# Autodesk Inventor assembly: v2_obstaculo
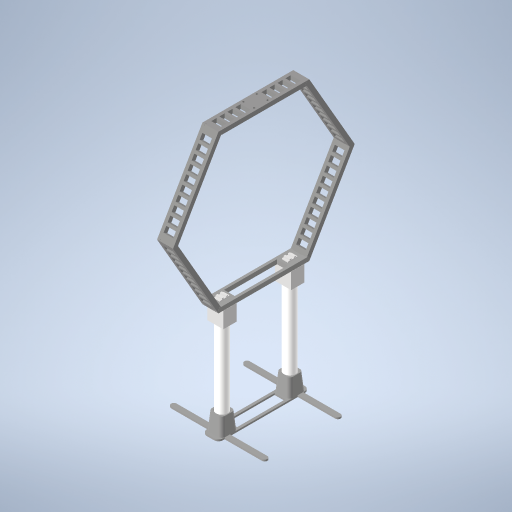
[picture p0: Inventor's stored thumbnail of the model, 512x512]
Saved by Autodesk Inventor 2024.3 (Build 283343000, 343)
## iProperties
Created: 2024-10-22
Part Number: v2_obstaculo
Document SubType Name: Assembly
Designer: pjcaa
Author: pjcaa
## Documents named in this file (8)
- C:\Users\pjcaa\Desktop\Educación\Semestres\5to año - Semestre 10\Diseño e innovación en ingeniería 2\Trabajo de graduacion\Archivos CAD\OBSTACULO_HEXAGONAL\ENSAMBLE_CON_EXTENSION.iam
- C:\Users\pjcaa\Desktop\Educación\Semestres\5to año - Semestre 10\Diseño e innovación en ingeniería 2\Trabajo de graduacion\Archivos CAD\OBSTACULO_HEXAGONAL\HEXAGONO_BASE.ipt
- C:\Users\pjcaa\Desktop\Educación\Semestres\5to año - Semestre 10\Diseño e innovación en ingeniería 2\Trabajo de graduacion\Archivos CAD\OBSTACULO_HEXAGONAL\EXTENSION_SOPORTE.ipt
- C:\Users\pjcaa\Desktop\Educación\Semestres\5to año - Semestre 10\Diseño e innovación en ingeniería 2\Trabajo de graduacion\Archivos CAD\OBSTACULO_HEXAGONAL\PIN.ipt
- C:\Users\pjcaa\Desktop\Educación\Semestres\5to año - Semestre 10\Diseño e innovación en ingeniería 2\Trabajo de graduacion\Archivos CAD\OBSTACULO_HEXAGONAL\EXTENSION_BASE.ipt
- C:\Users\pjcaa\Desktop\Educación\Semestres\5to año - Semestre 10\Diseño e innovación en ingeniería 2\Trabajo de graduacion\Archivos CAD\OBSTACULO_HEXAGONAL\HEXAGONO_LATERAL.ipt
- C:\Users\pjcaa\Desktop\Educación\Semestres\5to año - Semestre 10\Diseño e innovación en ingeniería 2\Trabajo de graduacion\Archivos CAD\OBSTACULO_HEXAGONAL\HEXGAONO_SUPERIOR.ipt
- C:\Users\pjcaa\Desktop\Educación\Semestres\5to año - Semestre 10\Diseño e innovación en ingeniería 2\Trabajo de graduacion\Archivos CAD\OBSTACULO_HEXAGONAL\TUBO.ipt
## Components (13 placed, 5 different names)
1. HEXAGONO_BASE:1 — Mate:1, Mate:2, Mate:3, Mate:4, Mate:5, Mate:10, Flush:7, Flush:8, Flush:9, Flush:10, Mate:11
2. sujetador_base:1 — Mate:1, Flush:1, Flush:2, Mate:2, Mate:6, Mate:7, Mate:14, Mate:18
3. sujetador_base:2 — Flush:1, Flush:2, Mate:3, Mate:4, Mate:13, Mate:19
4. sujetador_base:3 — Mate:5, Mate:6, Mate:7, Flush:14, Flush:15
5. EXTENSION_BASE:1 — Mate:13, Mate:14, Mate:15, Mate:16, Mate:17
6. HEXAGONO_LATERAL:1 — Mate:8, Flush:3, Flush:4, Flush:10, Mate:11
7. HEXGAONO_SUPERIOR:1 — Mate:12, Flush:11, Flush:12
8. HEXAGONO_LATERAL:2 — Mate:8, Flush:3, Flush:4, Flush:9, Mate:12, Flush:11
9. HEXAGONO_LATERAL:3 — Mate:10, Flush:7, Flush:8
10. HEXAGONO_LATERAL:4 — Flush:12
11. sujetador_base:4 — Mate:16, Flush:13, Mate:17, Mate:18
12. sujetador_base:5 — Mate:15, Flush:13
13. sujetador_base:6 — Flush:14, Flush:15, Mate:19
## Relationships (34: Mate 19, Flush 15)
- Mate:1: HEXAGONO_BASE:1 ↔ sujetador_base:1
- Flush:1: sujetador_base:1 ↔ sujetador_base:2
- Flush:2: sujetador_base:1 ↔ sujetador_base:2
- Mate:2: HEXAGONO_BASE:1 ↔ sujetador_base:1
- Mate:3: HEXAGONO_BASE:1 ↔ sujetador_base:2
- Mate:4: HEXAGONO_BASE:1 ↔ sujetador_base:2
- Mate:5: HEXAGONO_BASE:1 ↔ sujetador_base:3
- Mate:6: sujetador_base:1 ↔ sujetador_base:3
- Mate:7 (0.25 mm): sujetador_base:1 ↔ sujetador_base:3
- Mate:8: HEXAGONO_LATERAL:1 ↔ HEXAGONO_LATERAL:2
- Flush:3: HEXAGONO_LATERAL:1 ↔ HEXAGONO_LATERAL:2
- Flush:4: HEXAGONO_LATERAL:1 ↔ HEXAGONO_LATERAL:2
- [Mate]: HEXAGONO_LATERAL:3 ↔ HEXAGONO_LATERAL:4
- [Flush]: HEXAGONO_LATERAL:3 ↔ HEXAGONO_LATERAL:4
- [Flush]: HEXAGONO_LATERAL:3 ↔ HEXAGONO_LATERAL:4
- Mate:10: HEXAGONO_BASE:1 ↔ HEXAGONO_LATERAL:3
- Flush:7: HEXAGONO_BASE:1 ↔ HEXAGONO_LATERAL:3
- Flush:8: HEXAGONO_BASE:1 ↔ HEXAGONO_LATERAL:3
- Flush:9: HEXAGONO_BASE:1 ↔ HEXAGONO_LATERAL:2
- Flush:10: HEXAGONO_BASE:1 ↔ HEXAGONO_LATERAL:1
- Mate:11: HEXAGONO_BASE:1 ↔ HEXAGONO_LATERAL:1
- Mate:12: HEXGAONO_SUPERIOR:1 ↔ HEXAGONO_LATERAL:2
- Flush:11: HEXGAONO_SUPERIOR:1 ↔ HEXAGONO_LATERAL:2
- Flush:12: HEXGAONO_SUPERIOR:1 ↔ HEXAGONO_LATERAL:4
- Mate:13: sujetador_base:2 ↔ EXTENSION_BASE:1
- Mate:14: sujetador_base:1 ↔ EXTENSION_BASE:1
- Mate:15: EXTENSION_BASE:1 ↔ sujetador_base:5
- Mate:16: EXTENSION_BASE:1 ↔ sujetador_base:4
- Flush:13: sujetador_base:4 ↔ sujetador_base:5
- Mate:17: EXTENSION_BASE:1 ↔ sujetador_base:4
- Mate:18: sujetador_base:1 ↔ sujetador_base:4
- Flush:14: sujetador_base:3 ↔ sujetador_base:6
- Flush:15: sujetador_base:3 ↔ sujetador_base:6
- Mate:19: sujetador_base:2 ↔ sujetador_base:6
## Named parameters: d12_d9 = 0 mm, d13_d10 = 0 mm, d14_d11 = 0 mm
